# Autodesk Inventor assembly: AVT-PP-35
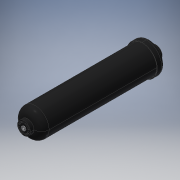
[picture p0: Inventor's stored thumbnail of the model, 180x180]
Saved by Autodesk Inventor 2016 SP2 (Build 200236200, 236)
## iProperties
Company: TraceParts S.A.
Created: 2016-10-27
Part Number: AVT-PP-35
Checked By: TraceParts S.A.
Catalog Web Link: www.traceparts.com
Description: Polypropylene Air Volume Tank, 35 Volume Cubic In. Max 125 PSI
Vendor: Clippard Minimatic
Document SubType Name: Assembly
Designer: TraceParts
Mass: 241.419 g
Surface Area: 1309.83 cm^2
Volume: 265.137 cm^3
Density: 0.910546 g/cm^3
REFERENCE: AVT-PP-35
SUPPLIER: Clippard Minimatic
DESIGN: Polypropylene Air Volume Tank, 35 Volume Cubic In. Max 125 PSI
OMNICLASS23: 23.27.33.00
TraceParts.PartVersion: 1.0.5
TraceParts.PartStatus: Published
TraceParts.PartNumber: 10-20022015-101355
TraceParts.PartLanguage: en
TraceParts.InstanceId: 10-20022015-10135589R27TA0FMO4CISB5QX8VZ8WO
TraceParts.PartTitle: Polypropylene Air Volume Tank
TRACEPARTS: TRACEPARTS
TraceParts.ClassPath: CLIPPARD:10-20022015-101355
Title: Polypropylene Air Volume Tank, 35 Volume Cubic In. Max 125 PSI
Author: TraceParts
## Documents named in this file (5)
- E:\GrabCAD\Power Hawks CAD\Pneumatic Resources\Clippard Air Tank\avt-pp-35.iam
- E:\GrabCAD\Power Hawks CAD\Pneumatic Resources\Clippard Air Tank\avt-pp-35_04.ipt
- E:\GrabCAD\Power Hawks CAD\Pneumatic Resources\Clippard Air Tank\avt-pp-35_03.ipt
- E:\GrabCAD\Power Hawks CAD\Pneumatic Resources\Clippard Air Tank\avt-pp-35_02.ipt
- E:\GrabCAD\Power Hawks CAD\Pneumatic Resources\Clippard Air Tank\avt-pp-35_01.ipt
## Components (4 placed, 4 different names)
1. avt-pp-35_04:1 — Rigid:1, Rotational:1
2. avt-pp-35_02:1 — Rigid:1, Rotational:2
3. avt-pp-35_03:1 — Rotational:1
4. avt-pp-35_01:1 — Rotational:2
## Relationships (3: RevoluteJoint 2, WeldJoint 1)
- Rigid:1 [WeldJoint]: avt-pp-35_04:1 ↔ avt-pp-35_02:1
- Rotational:1 [RevoluteJoint]: avt-pp-35_04:1 ↔ avt-pp-35_03:1
- Rotational:2 [RevoluteJoint]: avt-pp-35_02:1 ↔ avt-pp-35_01:1
